# Autodesk Inventor assembly: Evo
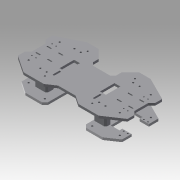
[picture p0: Inventor's stored thumbnail of the model, 180x180]
Saved by Autodesk Inventor 2016 (Build 200138000, 138)
## iProperties
Created: 2017-12-05
Part Number: Evo
Material: Générique
Document SubType Name: Assembly
Designer: LogOut
Author: LogOut
## Documents named in this file (4)
- C:\Travail\Objets\GitHub\Evo_Mechanical\Mechanic\Modelisation\Evo.iam
- C:\Travail\Objets\GitHub\Evo_Mechanical\Mechanic\Modelisation\Wheel_Support.ipt
- C:\Travail\Objets\GitHub\Evo_Mechanical\Mechanic\Modelisation\Motor_Support.ipt
- C:\Travail\Objets\GitHub\Evo_Mechanical\Mechanic\Modelisation\Wheel_Block.ipt
## Components (5 placed, 3 different names)
1. Motor_Support:1 — Placage:1, Placage:3, Placage:4, Placage:5, Placage:6, Placage:7, Placage:8, Placage:9
2. Wheel_Support:1 — Placage:3, Placage:8, Affleurement:1
3. Wheel_Support:2 — Placage:1, Placage:9, Affleurement:1
4. Wheel_Block:1 — Placage:4, Placage:6, Affleurement:2
5. Wheel_Block:2 — Placage:5, Placage:7, Affleurement:2
## Relationships (10: Mate 8, Flush 2)
- Placage:1 [Mate]: Motor_Support:1 ↔ Wheel_Support:2
- Placage:3 [Mate]: Motor_Support:1 ↔ Wheel_Support:1
- Placage:4 [Mate]: Motor_Support:1 ↔ Wheel_Block:1
- Placage:5 [Mate]: Motor_Support:1 ↔ Wheel_Block:2
- Placage:6 [Mate]: Motor_Support:1 ↔ Wheel_Block:1
- Placage:7 [Mate]: Motor_Support:1 ↔ Wheel_Block:2
- Placage:8 [Mate]: Motor_Support:1 ↔ Wheel_Support:1
- Placage:9 [Mate]: Motor_Support:1 ↔ Wheel_Support:2
- Affleurement:1 [Flush]: Wheel_Support:1 ↔ Wheel_Support:2
- Affleurement:2 [Flush]: Wheel_Block:1 ↔ Wheel_Block:2
